# Autodesk Inventor assembly: hip_joint
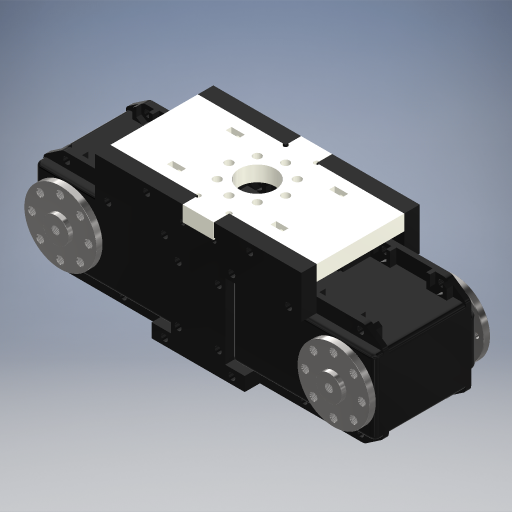
[picture p0: Inventor's stored thumbnail of the model, 512x512]
Saved by Autodesk Inventor 2024 (Build 280153000, 153)
## iProperties
Created: 2024-09-15
Part Number: hip_joint
Document SubType Name: Assembly
Designer: msi
Author: msi
## Documents named in this file (6)
- C:\Users\msi\GITHUB\19th_intern_kgh_fight_robot\부품\Lower_Body\Hip_joint\hip_joint.iam
- C:\Users\msi\GITHUB\19th_intern_kgh_fight_robot\부품\ROBOTIS(Inventor 2024 ver.)\다이나믹셀\MX-64T+idle.ipt.iam
- C:\Users\msi\GITHUB\19th_intern_kgh_fight_robot\부품\ROBOTIS(Inventor 2024 ver.)\혼\64-106Horn.ipt
- C:\Users\msi\GITHUB\19th_intern_kgh_fight_robot\부품\Lower_Body\Hip_joint\hip joint connection.ipt
- C:\Users\msi\GITHUB\19th_intern_kgh_fight_robot\부품\Lower_Body\Hip_joint\hip joint_body connection.ipt
- MX-64T+idle.ipt
## Components (7 placed, 4 different names)
1. MX-64T+idle.ipt:1 [sub-assembly] — 삽입:6, 삽입:7, 삽입:8, 삽입:13, 삽입:14
2. MX-64T+idle.ipt:2 [sub-assembly] — 삽입:5, 삽입:9, 삽입:10, 삽입:11, 삽입:12
3. 64-106Horn:1 — 삽입:5
4. 64-106Horn:2 — 삽입:6
5. hip joint connection:1 — 삽입:7, 삽입:8, 삽입:9, 삽입:10, 삽입:17, 삽입:18
6. hip joint connection:2 — 삽입:11, 삽입:12, 삽입:13, 삽입:14, 삽입:15, 삽입:16
7. hip joint_body connection:1 — 삽입:15, 삽입:16, 삽입:17, 삽입:18
## Relationships (14: Insert 14)
- 삽입:5 [Insert]: MX-64T+idle.ipt:2 ↔ 64-106Horn:1
- 삽입:6 [Insert]: MX-64T+idle.ipt:1 ↔ 64-106Horn:2
- 삽입:7 [Insert]: MX-64T+idle.ipt:1 ↔ hip joint connection:1
- 삽입:8 [Insert]: MX-64T+idle.ipt:1 ↔ hip joint connection:1
- 삽입:9 [Insert]: MX-64T+idle.ipt:2 ↔ hip joint connection:1
- 삽입:10 [Insert]: MX-64T+idle.ipt:2 ↔ hip joint connection:1
- 삽입:11 [Insert]: MX-64T+idle.ipt:2 ↔ hip joint connection:2
- 삽입:12 [Insert]: MX-64T+idle.ipt:2 ↔ hip joint connection:2
- 삽입:13 [Insert]: MX-64T+idle.ipt:1 ↔ hip joint connection:2
- 삽입:14 [Insert]: MX-64T+idle.ipt:1 ↔ hip joint connection:2
- 삽입:15 [Insert]: hip joint connection:2 ↔ hip joint_body connection:1
- 삽입:16 [Insert]: hip joint connection:2 ↔ hip joint_body connection:1
- 삽입:17 [Insert]: hip joint connection:1 ↔ hip joint_body connection:1
- 삽입:18 [Insert]: hip joint connection:1 ↔ hip joint_body connection:1
